# Autodesk Inventor assembly: Omni Roller 6 in
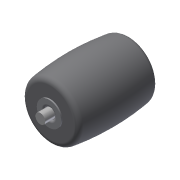
[picture p0: Inventor's stored thumbnail of the model, 180x180]
Saved by Autodesk Inventor 2013 (Build 170138000, 138)
## iProperties
Created: 2012-12-30
Part Number: Omni Roller 6 in
Document SubType Name: Assembly
Designer: Nemo
Author: Nemo
## Documents named in this file (4)
- H:\Nemo\Documents\Robotics\VexPro\Omni Wheel\Components\Omni Roller 6 in.iam
- H:\Nemo\Documents\Robotics\VexPro\Omni Wheel\Components\Omni Roller Shaft 6 in.ipt
- H:\Nemo\Documents\Robotics\VexPro\Omni Wheel\Components\Omni Wheel Roller 6 in.ipt
- H:\Nemo\Documents\Robotics\VexPro\Omni Wheel\Components\Omni Roller Bearing.ipt
## Components (4 placed, 3 different names)
1. Omni Roller Shaft 6 in:1
2. Omni Wheel Roller 6 in:1
3. Omni Roller Bearing:1
4. Omni Roller Bearing:2
## Relationships (4: Insert 2, Mate 2)
- [Insert]: Omni Wheel Roller 6 in:1 ↔ Omni Roller Bearing:2
- [Insert]: Omni Wheel Roller 6 in:1 ↔ Omni Roller Bearing:1
- [Mate]: Omni Roller Shaft 6 in:1 ↔ Omni Wheel Roller 6 in:1
- [Mate]: Omni Roller Shaft 6 in:1 ↔ Omni Wheel Roller 6 in:1
